# Autodesk Inventor assembly: 42146-37
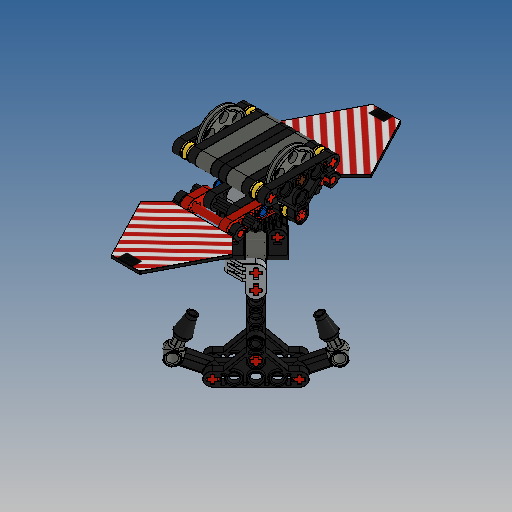
[picture p0: Inventor's stored thumbnail of the model, 512x512]
Saved by Autodesk Inventor 2025.1 (Build 291241000, 241)
## iProperties
Created: 2024-12-15
Part Number: 42146-37
Material: Generisch
Document SubType Name: Assembly
Designer: hp.muther
Author: hp.muther
## Documents named in this file (25)
- D:\Inventor\Projekte\Muther\LEGO Technic\LEGO Technik - Raupenkran LR 13000 (42146)\42146-37.iam
- D:\Inventor\Projekte\Muther\LEGO Technic\LEGO Pieces\Achsen\4519-LtBluishGray.ipt
- D:\Inventor\Projekte\Muther\LEGO Technic\LEGO Pieces\Verbindungselemente\32016-Black.ipt
- D:\Inventor\Projekte\Muther\LEGO Technic\LEGO Pieces\Verbindungselemente mit Pin\10197-DkBluishGray.ipt
- D:\Inventor\Projekte\Muther\LEGO Technic\LEGO Pieces\Steine rund\59900-Black.ipt
- D:\Inventor\Projekte\Muther\LEGO Technic\LEGO Pieces\Achsen\32062-Red.ipt
- D:\Inventor\Projekte\Muther\LEGO Technic\LEGO Pieces\Rahmen, T-Stücke\99773-Black.ipt
- D:\Inventor\Projekte\Muther\LEGO Technic\LEGO Pieces\Lochbalken schmal\11478-Black.ipt
- D:\Inventor\Projekte\Muther\LEGO Technic\LEGO Pieces\Pin's\2780-Black.ipt
- D:\Inventor\Projekte\Muther\LEGO Technic\LEGO Pieces\Verbindungselemente\92907-LtBluishGray.ipt
- D:\Inventor\Projekte\Muther\LEGO Technic\LEGO Pieces\Verbindungselemente\41678-Black.ipt
- D:\Inventor\Projekte\Muther\LEGO Technic\LEGO Pieces\Verbindungselemente\32291-DkBluishGray.ipt
- D:\Inventor\Projekte\Muther\LEGO Technic\LEGO Pieces\Pin's\6558-Blue.ipt
- D:\Inventor\Projekte\Muther\LEGO Technic\LEGO Pieces\Zahnrad\99009-LtBluishGray.ipt
- D:\Inventor\Projekte\Muther\LEGO Technic\LEGO Pieces\Zahnrad\99010-Black.ipt
- D:\Inventor\Projekte\Muther\LEGO Technic\LEGO Pieces\Lochbalken schmal\32449-Red.ipt
- D:\Inventor\Projekte\Muther\LEGO Technic\LEGO Pieces\Lochbalken schmal\41677-Red.ipt
- D:\Inventor\Projekte\Muther\LEGO Technic\LEGO Pieces\Achsen\3705-Black.ipt
- D:\Inventor\Projekte\Muther\LEGO Technic\LEGO Pieces\Achsen\21462-Red.ipt
- D:\Inventor\Projekte\Muther\LEGO Technic\LEGO Pieces\Achsen\24316-ReddishBrown.ipt
- D:\Inventor\Projekte\Muther\LEGO Technic\LEGO Pieces\Achsen\3706-Red.ipt
- D:\Inventor\Projekte\Muther\LEGO Technic\LEGO Pieces\Lochbalken\32316-DkBluishGray.ipt
- D:\Inventor\Projekte\Muther\LEGO Technic\LEGO Pieces\Rund\4265c-Yellow.ipt
- D:\Inventor\Projekte\Muther\LEGO Technic\LEGO Pieces\Räder, Raupe\4185-DkBluishGray.ipt
- D:\Inventor\Projekte\Muther\LEGO Technic\LEGO Technik - Raupenkran LR 13000 (42146)\42146_53913_1.ipt
## Components (64 placed, 24 different names)
1. 4519-LtBluishGray:1 — Einfügen:1, Einfügen:6, Passend:3
2. 32016-Black:1 — Einfügen:1, Einfügen:2, Passend:1, Passend:4
3. 10197-DkBluishGray:1 — Einfügen:2, Einfügen:3, Passend:1
4. 59900-Black:1 — Einfügen:3
5. 32016-Black:2 — Einfügen:6, Passend:3, Einfügen:9, Einfügen:14
6. 10197-DkBluishGray:2
7. 59900-Black:2
8. 32062-Red:1 — Einfügen:7, Passend:4, Passend:5
9. 32062-Red:2 — Einfügen:8
10. 99773-Black:1 — Einfügen:7, Einfügen:8, Einfügen:9, Einfügen:13
11. 99773-Black:2 — Einfügen:14, Passend:5
12. 32062-Red:3 — Einfügen:10
13. 11478-Black:1 — Einfügen:10, Einfügen:11, Einfügen:12, Einfügen:13
14. 11478-Black:2 — Einfügen:12, Einfügen:16, Passend:6
15. 2780-Black:1 — Einfügen:11
16. 32062-Red:4 — Einfügen:15, Passend:6
17. 92907-LtBluishGray:1 — Einfügen:15, Einfügen:16, Einfügen:25, Einfügen:26
18. 41678-Black:1 — Einfügen:17, Einfügen:21, Passend:8
19. 32291-DkBluishGray:1 — Einfügen:18, Einfügen:19, Einfügen:21, Einfügen:22, Einfügen:25
20. 6558-Blue:1 — Einfügen:19, Passend:8
21. 6558-Blue:2 — Einfügen:18, Passend:7
22. 99009-LtBluishGray:1 — Einfügen:24, Einfügen:27, Einfügen:28, Einfügen:29, Einfügen:30
23. 99010-Black:1 — Einfügen:23, Passend:9, Einfügen:24
24. 32062-Red:5 — Einfügen:17, Passend:9
25. 41678-Black:2 — Einfügen:22, Passend:7, Einfügen:23
26. 32062-Red:6
27. 32062-Red:7 — Einfügen:26
28. 11478-Black:3 — Einfügen:29, Passend:10, Einfügen:38, Passend:12, Passend:13, Winkel:1
29. 6558-Blue:3 — Einfügen:28
30. 6558-Blue:4 — Einfügen:27, Passend:10, Passend:11
31. 11478-Black:4 — Einfügen:30, Passend:11, Einfügen:37
32. 32449-Red:1 — Einfügen:31, Einfügen:32, Einfügen:38, Einfügen:54, Einfügen:55, Einfügen:63
33. 41677-Red:1 — Einfügen:33
34. 3705-Black:1 — Einfügen:32, Einfügen:33, Passend:12
35. 21462-Red:1 — Einfügen:31
36. 32449-Red:2 — Einfügen:37, Einfügen:62
37. 41677-Red:2
38. 3705-Black:2 — Passend:13
39. 21462-Red:2
40. 99773-Black:3 — Einfügen:42, Einfügen:43, Passend:14, Einfügen:44, Einfügen:45, Einfügen:46
41. 6558-Blue:5 — Einfügen:39
42. 6558-Blue:6 — Einfügen:40
43. 24316-ReddishBrown:1 — Einfügen:41, Einfügen:58
44. 24316-ReddishBrown:2 — Einfügen:42, Einfügen:59
45. 3706-Red:1 — Einfügen:44, Passend:15, Passend:16, Passend:18, Passend:21
46. 3706-Red:2 — Einfügen:45, Passend:17, Passend:22
47. 32316-DkBluishGray:1 — Einfügen:46, Passend:15, Einfügen:53
48. 99773-Black:4 — Einfügen:39, Einfügen:40, Einfügen:41, Einfügen:43, Passend:14, Einfügen:48, Winkel:1
49. 99773-Black:5 — Einfügen:47, Passend:16, Einfügen:49, Einfügen:50, Fluchtend:1, Fluchtend:2, Einfügen:54, Einfügen:56
50. 32316-DkBluishGray:2 — Einfügen:47, Einfügen:48, Passend:17
51. 4265c-Yellow:1 — Einfügen:50, Fluchtend:1, Einfügen:61
52. 4265c-Yellow:2 — Einfügen:49, Fluchtend:2
53. 99773-Black:6 — Einfügen:53, Passend:18, Einfügen:57
54. 4265c-Yellow:3 — Einfügen:60
55. 4265c-Yellow:4
56. 3706-Red:3 — Einfügen:55, Passend:19, Passend:20
57. 4265c-Yellow:5 — Einfügen:56, Passend:19
58. 4265c-Yellow:6 — Einfügen:57, Passend:20
59. 4185-DkBluishGray:1 — Einfügen:58
60. 4185-DkBluishGray:2 — Einfügen:59
61. 99773-Black:7 — Einfügen:61, Passend:21
62. 99773-Black:8 — Einfügen:60, Passend:22
63. 42146_53913_1:1 — Einfügen:63, Fluchtend:5
64. 42146_53913_1:2 — Einfügen:62, Fluchtend:5
## Relationships (91: Insert 63, Mate 22, Flush 5, Angle 1)
- Einfügen:1 [Insert] (-8 mm): 4519-LtBluishGray:1 ↔ 32016-Black:1
- Einfügen:2 [Insert]: 32016-Black:1 ↔ 10197-DkBluishGray:1
- Einfügen:3 [Insert]: 10197-DkBluishGray:1 ↔ 59900-Black:1
- Passend:1 [Mate]: 32016-Black:1 ↔ 10197-DkBluishGray:1
- [Insert]: 32016-Black:2 ↔ 10197-DkBluishGray:2
- [Insert]: 10197-DkBluishGray:2 ↔ 59900-Black:2
- [Mate]: 32016-Black:2 ↔ 10197-DkBluishGray:2
- Einfügen:6 [Insert] (-8 mm): 4519-LtBluishGray:1 ↔ 32016-Black:2
- Passend:3 [Mate]: 4519-LtBluishGray:1 ↔ 32016-Black:2
- Einfügen:7 [Insert]: 32062-Red:1 ↔ 99773-Black:1
- Einfügen:8 [Insert]: 32062-Red:2 ↔ 99773-Black:1
- Einfügen:9 [Insert]: 32016-Black:2 ↔ 99773-Black:1
- Passend:4 [Mate]: 32016-Black:1 ↔ 32062-Red:1
- Einfügen:10 [Insert] (-8 mm): 32062-Red:3 ↔ 11478-Black:1
- Einfügen:11 [Insert]: 11478-Black:1 ↔ 2780-Black:1
- Einfügen:12 [Insert]: 11478-Black:1 ↔ 11478-Black:2
- Einfügen:13 [Insert]: 99773-Black:1 ↔ 11478-Black:1
- Einfügen:14 [Insert]: 32016-Black:2 ↔ 99773-Black:2
- Passend:5 [Mate]: 32062-Red:1 ↔ 99773-Black:2
- Einfügen:15 [Insert]: 32062-Red:4 ↔ 92907-LtBluishGray:1
- Einfügen:16 [Insert]: 11478-Black:2 ↔ 92907-LtBluishGray:1
- Passend:6 [Mate]: 11478-Black:2 ↔ 32062-Red:4
- Einfügen:17 [Insert]: 41678-Black:1 ↔ 32062-Red:5
- Einfügen:18 [Insert]: 32291-DkBluishGray:1 ↔ 6558-Blue:2
- Einfügen:19 [Insert]: 32291-DkBluishGray:1 ↔ 6558-Blue:1
- [Insert]: 41678-Black:2 ↔ 32062-Red:6
- Einfügen:21 [Insert]: 41678-Black:1 ↔ 32291-DkBluishGray:1
- Einfügen:22 [Insert]: 32291-DkBluishGray:1 ↔ 41678-Black:2
- Passend:7 [Mate]: 6558-Blue:2 ↔ 41678-Black:2
- Passend:8 [Mate]: 41678-Black:1 ↔ 6558-Blue:1
- Einfügen:23 [Insert]: 99010-Black:1 ↔ 41678-Black:2
- Passend:9 [Mate]: 99010-Black:1 ↔ 32062-Red:5
- Einfügen:24 [Insert]: 99009-LtBluishGray:1 ↔ 99010-Black:1
- Einfügen:25 [Insert]: 92907-LtBluishGray:1 ↔ 32291-DkBluishGray:1
- Einfügen:26 [Insert]: 92907-LtBluishGray:1 ↔ 32062-Red:7
- Einfügen:27 [Insert]: 99009-LtBluishGray:1 ↔ 6558-Blue:4
- Einfügen:28 [Insert]: 99009-LtBluishGray:1 ↔ 6558-Blue:3
- Einfügen:29 [Insert]: 99009-LtBluishGray:1 ↔ 11478-Black:3
- Einfügen:30 [Insert]: 99009-LtBluishGray:1 ↔ 11478-Black:4
- Passend:10 [Mate]: 11478-Black:3 ↔ 6558-Blue:4
- Passend:11 [Mate]: 6558-Blue:4 ↔ 11478-Black:4
- Einfügen:31 [Insert] (-8 mm): 32449-Red:1 ↔ 21462-Red:1
- Einfügen:32 [Insert] (-8 mm): 32449-Red:1 ↔ 3705-Black:1
- Einfügen:33 [Insert] (-8 mm): 41677-Red:1 ↔ 3705-Black:1
- [Insert] (-8 mm): 32449-Red:2 ↔ 21462-Red:2
- [Insert] (-8 mm): 32449-Red:2 ↔ 3705-Black:2
- [Insert] (-8 mm): 41677-Red:2 ↔ 3705-Black:2
- Einfügen:37 [Insert]: 11478-Black:4 ↔ 32449-Red:2
- Einfügen:38 [Insert]: 11478-Black:3 ↔ 32449-Red:1
- Passend:12 [Mate]: 11478-Black:3 ↔ 3705-Black:1
- Passend:13 [Mate]: 11478-Black:3 ↔ 3705-Black:2
- Einfügen:39 [Insert]: 6558-Blue:5 ↔ 99773-Black:4
- Einfügen:40 [Insert]: 6558-Blue:6 ↔ 99773-Black:4
- Einfügen:41 [Insert]: 24316-ReddishBrown:1 ↔ 99773-Black:4
- Einfügen:42 [Insert]: 99773-Black:3 ↔ 24316-ReddishBrown:2
- Einfügen:43 [Insert]: 99773-Black:3 ↔ 99773-Black:4
- Passend:14 [Mate]: 99773-Black:3 ↔ 99773-Black:4
- Einfügen:44 [Insert] (-28 mm): 99773-Black:3 ↔ 3706-Red:1
- Einfügen:45 [Insert] (-28 mm): 99773-Black:3 ↔ 3706-Red:2
- Einfügen:46 [Insert]: 99773-Black:3 ↔ 32316-DkBluishGray:1
- Passend:15 [Mate]: 3706-Red:1 ↔ 32316-DkBluishGray:1
- Einfügen:47 [Insert]: 99773-Black:5 ↔ 32316-DkBluishGray:2
- Einfügen:48 [Insert]: 99773-Black:4 ↔ 32316-DkBluishGray:2
- Passend:16 [Mate]: 3706-Red:1 ↔ 99773-Black:5
- Passend:17 [Mate]: 3706-Red:2 ↔ 32316-DkBluishGray:2
- Einfügen:49 [Insert]: 99773-Black:5 ↔ 4265c-Yellow:2
- Einfügen:50 [Insert]: 99773-Black:5 ↔ 4265c-Yellow:1
- Fluchtend:1 [Flush]: 99773-Black:5 ↔ 4265c-Yellow:1
- Fluchtend:2 [Flush]: 99773-Black:5 ↔ 4265c-Yellow:2
- [Insert]: 99773-Black:6 ↔ 4265c-Yellow:4
- [Insert]: 99773-Black:6 ↔ 4265c-Yellow:3
- [Flush]: 99773-Black:6 ↔ 4265c-Yellow:3
- [Flush]: 99773-Black:6 ↔ 4265c-Yellow:4
- Einfügen:53 [Insert]: 32316-DkBluishGray:1 ↔ 99773-Black:6
- Passend:18 [Mate]: 3706-Red:1 ↔ 99773-Black:6
- Einfügen:54 [Insert]: 32449-Red:1 ↔ 99773-Black:5
- Einfügen:55 [Insert] (-36 mm): 32449-Red:1 ↔ 3706-Red:3
- Einfügen:56 [Insert]: 99773-Black:5 ↔ 4265c-Yellow:5
- Passend:19 [Mate]: 3706-Red:3 ↔ 4265c-Yellow:5
- Einfügen:57 [Insert]: 99773-Black:6 ↔ 4265c-Yellow:6
- Passend:20 [Mate]: 3706-Red:3 ↔ 4265c-Yellow:6
- Winkel:1 [Angle] (0 deg): 11478-Black:3 ↔ 99773-Black:4
- Einfügen:58 [Insert] (-8 mm): 24316-ReddishBrown:1 ↔ 4185-DkBluishGray:1
- Einfügen:59 [Insert] (-8 mm): 24316-ReddishBrown:2 ↔ 4185-DkBluishGray:2
- Einfügen:60 [Insert]: 4265c-Yellow:3 ↔ 99773-Black:8
- Einfügen:61 [Insert]: 4265c-Yellow:1 ↔ 99773-Black:7
- Passend:21 [Mate]: 3706-Red:1 ↔ 99773-Black:7
- Passend:22 [Mate]: 3706-Red:2 ↔ 99773-Black:8
- Einfügen:62 [Insert] (0.8 mm): 32449-Red:2 ↔ 42146_53913_1:2
- Einfügen:63 [Insert] (0.8 mm): 32449-Red:1 ↔ 42146_53913_1:1
- Fluchtend:5 [Flush]: 42146_53913_1:1 ↔ 42146_53913_1:2
## Named parameters: d4_d1 = 0 mm, d5_d2 = 0 mm, d6_d3 = 0 mm, d25_d22 = 0 mm, d44_d41 = -8 mm, d45_d42 = -8 mm, d46_d43 = -8 mm, d61_d59 = 0 mm, d69_d65 = 0 mm, d70_d66 = 0 mm, d71_d67 = 0 mm, d72_d68 = 0 mm
